# Autodesk Inventor assembly: sail(open)
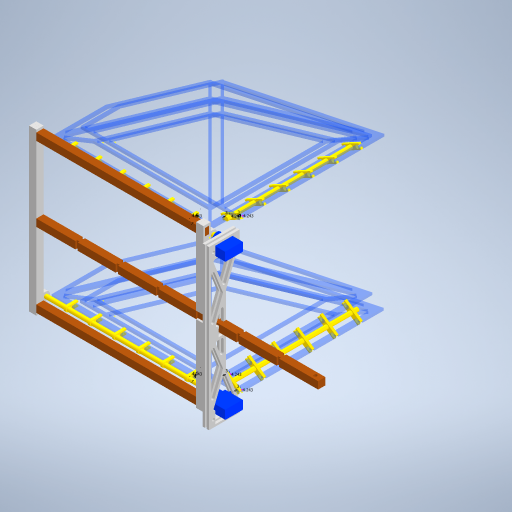
[picture p0: Inventor's stored thumbnail of the model, 512x512]
Saved by Autodesk Inventor 2024 (Build 280153000, 153)
## iProperties
Created: 2024-04-09
Part Number: sail(open)
Document SubType Name: Assembly
Designer: USER
Author: USER
## Documents named in this file (13)
- E:\university\大三\大三下\機工實務\圖檔\DesignVer2\sail(open).iam
- E:\university\大三\大三下\機工實務\圖檔\DesignVer2\main_Bar.ipt
- E:\university\大三\大三下\機工實務\圖檔\DesignVer2\main_Bar_3.ipt
- E:\university\大三\大三下\機工實務\圖檔\DesignVer2\Lower_Bar.ipt
- E:\university\大三\大三下\機工實務\圖檔\DesignVer2\upper_Bar.ipt
- E:\university\大三\大三下\機工實務\圖檔\DesignVer2\upper_Bar_3.ipt
- E:\university\大三\大三下\機工實務\圖檔\DesignVer2\side_Bar.ipt
- E:\university\大三\大三下\機工實務\圖檔\DesignVer2\[3DP]bar.ipt
- E:\university\大三\大三下\機工實務\圖檔\DesignVer2\Servo Motor SG90.ipt
- E:\university\大三\大三下\機工實務\圖檔\DesignVer2\side_motor.ipt
- E:\university\大三\大三下\機工實務\圖檔\DesignVer2\side_sail.ipt
- E:\university\大三\大三下\機工實務\圖檔\DesignVer2\[3DP]double_bar.ipt
- E:\university\大三\大三下\機工實務\圖檔\DesignVer2\side_sail_2.ipt
## Components (27 placed, 12 different names)
1. main_Bar:1 — 齊平:1, 齊平:2, 貼合:2, 貼合:7, 貼合:11
2. main_Bar:2 — 齊平:1, 齊平:2, 齊平:3, 齊平:4, 貼合:1, 貼合:2, 貼合:5, 貼合:6
3. main_Bar_3:1 — 齊平:3, 齊平:4, 貼合:1, 貼合:10, 齊平:13
4. Lower_Bar:1 — 齊平:5, 貼合:4, 齊平:8, 角度:1
5. Lower_Bar:2 — 齊平:5, 齊平:6, 貼合:3, 貼合:4, 齊平:7, 齊平:8, 貼合:28
6. upper_Bar:1 — 貼合:9, 齊平:10, 齊平:11, 貼合:10, 貼合:26
7. upper_Bar:2 — 貼合:8, 貼合:9, 齊平:9, 齊平:10, 齊平:11, 齊平:12, 齊平:13
8. upper_Bar_3:1 — 貼合:8, 齊平:9, 齊平:12, 貼合:11, 貼合:25, 貼合:27
9. Lower_Bar:3 — 齊平:6, 貼合:3, 齊平:7, 貼合:5, 貼合:6, 貼合:7, 貼合:16, 貼合:17, 貼合:18, 貼合:19, 貼合:20, 貼合:21, 角度:2
10. side_Bar:1 — 貼合:12, 齊平:14, 齊平:17, 貼合:21, 角度:6
11. side_Bar:2 — 貼合:12, 貼合:13, 齊平:14, 齊平:15, 齊平:16, 齊平:17, 貼合:20
12. side_Bar:3 — 貼合:13, 齊平:15, 齊平:16, 貼合:19
13. side_Bar:4 — 齊平:18, 齊平:20, 貼合:14
14. side_Bar:5 — 齊平:18, 齊平:19, 齊平:20, 齊平:21, 貼合:14, 貼合:15, 貼合:16, 貼合:18
15. side_Bar:6 — 齊平:19, 齊平:21, 貼合:15, 貼合:17, 角度:5
16. [3DP]bar:1 — 貼合:24, 貼合:25, 貼合:26, 貼合:29, 貼合:36, 貼合:37, 貼合:38
17. [3DP]bar:2 — 貼合:27, 貼合:28, 貼合:30, 貼合:31, 貼合:39, 貼合:40, 貼合:41
18. Servo Motor SG90:1 — 貼合:30, 貼合:31, 角度:2, 貼合:32, 貼合:33, 貼合:34, 貼合:35
19. Servo Motor SG90:2 — 貼合:24, 貼合:29, 角度:1
20. side_motor:1 — 貼合:32, 貼合:33, 貼合:34, 齊平:22, 齊平:23
21. side_motor:2 — 齊平:22, 齊平:23, 貼合:35
22. side_sail:1 — 貼合:36, 貼合:37, 貼合:38, 貼合:45, 貼合:46, 角度:6, 角度:8
23. side_sail:2 — 貼合:39, 貼合:40, 貼合:41, 貼合:42, 角度:4, 貼合:43, 齊平:24, 角度:5, 角度:7
24. [3DP]double_bar:1 — 貼合:45, 貼合:46, 貼合:47, 貼合:48
25. [3DP]double_bar:2 — 貼合:42, 角度:4, 貼合:43, 貼合:44
26. side_sail_2:1 — 齊平:24, 貼合:44, 角度:7
27. side_sail_2:2 — 貼合:47, 貼合:48, 角度:8
## Relationships (77: Mate 46, Flush 24, Angle 7)
- 齊平:1 [Flush]: main_Bar:1 ↔ main_Bar:2
- 齊平:2 [Flush]: main_Bar:1 ↔ main_Bar:2
- 齊平:3 [Flush]: main_Bar:2 ↔ main_Bar_3:1
- 齊平:4 [Flush]: main_Bar:2 ↔ main_Bar_3:1
- 貼合:1 [Mate]: main_Bar:2 ↔ main_Bar_3:1
- 貼合:2 [Mate]: main_Bar:1 ↔ main_Bar:2
- 齊平:5 [Flush]: Lower_Bar:1 ↔ Lower_Bar:2
- 齊平:6 [Flush]: Lower_Bar:2 ↔ Lower_Bar:3
- 貼合:3 [Mate]: Lower_Bar:2 ↔ Lower_Bar:3
- 貼合:4 [Mate]: Lower_Bar:1 ↔ Lower_Bar:2
- 齊平:7 [Flush]: Lower_Bar:2 ↔ Lower_Bar:3
- 齊平:8 [Flush]: Lower_Bar:1 ↔ Lower_Bar:2
- 貼合:5 [Mate]: main_Bar:2 ↔ Lower_Bar:3
- 貼合:6 [Mate]: main_Bar:2 ↔ Lower_Bar:3
- 貼合:7 [Mate]: main_Bar:1 ↔ Lower_Bar:3
- 貼合:8 [Mate]: upper_Bar:2 ↔ upper_Bar_3:1
- 貼合:9 [Mate]: upper_Bar:1 ↔ upper_Bar:2
- 齊平:9 [Flush]: upper_Bar:2 ↔ upper_Bar_3:1
- 齊平:10 [Flush]: upper_Bar:1 ↔ upper_Bar:2
- 齊平:11 [Flush]: upper_Bar:1 ↔ upper_Bar:2
- 齊平:12 [Flush]: upper_Bar:2 ↔ upper_Bar_3:1
- 貼合:10 [Mate]: main_Bar_3:1 ↔ upper_Bar:1
- 齊平:13 [Flush]: main_Bar_3:1 ↔ upper_Bar:2
- 貼合:11 [Mate]: main_Bar:1 ↔ upper_Bar_3:1
- 貼合:12 [Mate]: side_Bar:1 ↔ side_Bar:2
- 貼合:13 [Mate]: side_Bar:2 ↔ side_Bar:3
- 齊平:14 [Flush]: side_Bar:1 ↔ side_Bar:2
- 齊平:15 [Flush]: side_Bar:2 ↔ side_Bar:3
- 齊平:16 [Flush]: side_Bar:2 ↔ side_Bar:3
- 齊平:17 [Flush]: side_Bar:1 ↔ side_Bar:2
- 齊平:18 [Flush]: side_Bar:4 ↔ side_Bar:5
- 齊平:19 [Flush]: side_Bar:5 ↔ side_Bar:6
- 齊平:20 [Flush]: side_Bar:4 ↔ side_Bar:5
- 齊平:21 [Flush]: side_Bar:5 ↔ side_Bar:6
- 貼合:14 [Mate]: side_Bar:4 ↔ side_Bar:5
- 貼合:15 [Mate]: side_Bar:5 ↔ side_Bar:6
- 貼合:16 [Mate]: Lower_Bar:3 ↔ side_Bar:5
- 貼合:17 [Mate]: Lower_Bar:3 ↔ side_Bar:6
- 貼合:18 [Mate]: Lower_Bar:3 ↔ side_Bar:5
- 貼合:19 [Mate]: Lower_Bar:3 ↔ side_Bar:3
- 貼合:20 [Mate]: Lower_Bar:3 ↔ side_Bar:2
- 貼合:21 [Mate]: Lower_Bar:3 ↔ side_Bar:1
- 貼合:24 [Mate]: [3DP]bar:1 ↔ Servo Motor SG90:2
- 貼合:25 [Mate]: upper_Bar_3:1 ↔ [3DP]bar:1
- 貼合:26 [Mate]: upper_Bar:1 ↔ [3DP]bar:1
- 貼合:27 [Mate]: upper_Bar_3:1 ↔ [3DP]bar:2
- 貼合:28 [Mate]: Lower_Bar:2 ↔ [3DP]bar:2
- 貼合:29 [Mate]: [3DP]bar:1 ↔ Servo Motor SG90:2
- 貼合:30 [Mate]: [3DP]bar:2 ↔ Servo Motor SG90:1
- 貼合:31 [Mate]: [3DP]bar:2 ↔ Servo Motor SG90:1
- 角度:1 [Angle] (0 deg): Lower_Bar:1 ↔ Servo Motor SG90:2
- 角度:2 [Angle] (0 deg): Lower_Bar:3 ↔ Servo Motor SG90:1
- 貼合:32 [Mate]: Servo Motor SG90:1 ↔ side_motor:1
- 貼合:33 [Mate]: Servo Motor SG90:1 ↔ side_motor:1
- 貼合:34 [Mate]: Servo Motor SG90:1 ↔ side_motor:1
- 齊平:22 [Flush]: side_motor:1 ↔ side_motor:2
- 齊平:23 [Flush]: side_motor:1 ↔ side_motor:2
- 貼合:35 [Mate]: Servo Motor SG90:1 ↔ side_motor:2
- 貼合:36 [Mate]: [3DP]bar:1 ↔ side_sail:1
- 貼合:37 [Mate]: [3DP]bar:1 ↔ side_sail:1
- 貼合:38 [Mate]: [3DP]bar:1 ↔ side_sail:1
- 貼合:39 [Mate]: [3DP]bar:2 ↔ side_sail:2
- 貼合:40 [Mate]: [3DP]bar:2 ↔ side_sail:2
- 貼合:41 [Mate]: [3DP]bar:2 ↔ side_sail:2
- 貼合:42 [Mate]: side_sail:2 ↔ [3DP]double_bar:2
- 角度:4 [Angle] (0 deg): side_sail:2 ↔ [3DP]double_bar:2
- 貼合:43 [Mate]: side_sail:2 ↔ [3DP]double_bar:2
- 齊平:24 [Flush]: side_sail:2 ↔ side_sail_2:1
- 貼合:44 [Mate]: [3DP]double_bar:2 ↔ side_sail_2:1
- 貼合:45 [Mate]: side_sail:1 ↔ [3DP]double_bar:1
- 貼合:46 [Mate]: side_sail:1 ↔ [3DP]double_bar:1
- 貼合:47 [Mate]: [3DP]double_bar:1 ↔ side_sail_2:2
- 貼合:48 [Mate]: [3DP]double_bar:1 ↔ side_sail_2:2
- 角度:5 [Angle] (0 deg): side_Bar:6 ↔ side_sail:2
- 角度:6 [Angle] (0 deg): side_Bar:1 ↔ side_sail:1
- 角度:7 [Angle] (0 deg): side_sail:2 ↔ side_sail_2:1
- 角度:8 [Angle] (0 deg): side_sail:1 ↔ side_sail_2:2
